# Autodesk Inventor assembly: Bearing_Holder(t2.5)-8
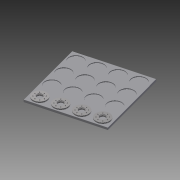
[picture p0: Inventor's stored thumbnail of the model, 180x180]
Saved by Autodesk Inventor 2013 (Build 170138000, 138)
## iProperties
Created: 2014-04-22
Part Number: Bearing_Holder(t2.5)-8
Document SubType Name: Assembly
Designer: andou
Author: andou
## Documents named in this file (3)
- C:\Users\andou\Documents\GitHub\Robotics-Project\design\RoboticsProject\project_4\cnc_data\Bearing_Holder(t2.5)-8.iam
- C:\Users\andou\Documents\GitHub\Robotics-Project\design\RoboticsProject\project_4\cnc_data\Bearing_Holder(t2.5).ipt
- C:\Users\andou\Documents\GitHub\Robotics-Project\design\RoboticsProject\project_4\cnc_data\fai20_sikiita.ipt
## Components (5 placed, 2 different names)
1. fai20_sikiita:1 — 挿入:1
2. Bearing_Holder(t2.5):1 — 挿入:1
3. Bearing_Holder(t2.5):2
4. Bearing_Holder(t2.5):3
5. Bearing_Holder(t2.5):4
## Component patterns: (4 elements, first: Bearing_Holder(t2.5):1)
## Relationships (1: Insert 1)
- 挿入:1 [Insert]: fai20_sikiita:1 ↔ Bearing_Holder(t2.5):1
